# Autodesk Inventor assembly: JigAssembly
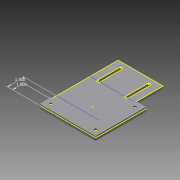
[picture p0: Inventor's stored thumbnail of the model, 180x180]
Saved by Autodesk Inventor 2014 (Build 180170000, 170)
## iProperties
Created: 2014-10-04
Part Number: JigAssembly
Document SubType Name: Assembly
Designer: Rachel
Author: Rachel
## Documents named in this file (3)
- C:\Users\Rachel\Desktop\PiE\Reflow Structure Inventor\JigAssembly.iam
- C:\Users\Rachel\Desktop\PiE\Reflow Structure Inventor\bottomLayer.ipt
- C:\Users\Rachel\Desktop\PiE\Reflow Structure Inventor\topLayer.ipt
## Components (2 placed, 2 different names)
1. bottomLayer:1 — Mate:1, Mate:2, Flush:1
2. topLayer:1 — Mate:1, Mate:2, Flush:1
## Relationships (3: Mate 2, Flush 1)
- Mate:1: bottomLayer:1 ↔ topLayer:1
- Mate:2: bottomLayer:1 ↔ topLayer:1
- Flush:1: bottomLayer:1 ↔ topLayer:1
